# Autodesk Inventor assembly: Hinge
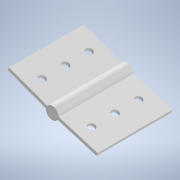
[picture p0: Inventor's stored thumbnail of the model, 180x180]
Saved by Autodesk Inventor 2020 (Build 240168000, 168)
## iProperties
Created: 2021-11-11
Part Number: Hinge
Document SubType Name: Assembly
Designer: 17185
Author: 17185
## Documents named in this file (3)
- C:\Users\17185\Desktop\chassis draft\Hinge\Hinge.iam
- C:\Users\17185\Desktop\chassis draft\Hinge\leaf.ipt
- C:\Users\17185\Desktop\chassis draft\Hinge\Pin.ipt
## Components (3 placed, 2 different names)
1. leaf:1 — Mate:1, Flush:1
2. leaf:2 — Flush:2, Mate:2
3. Pin:1 — Mate:1, Flush:1, Flush:2, Mate:2
## Relationships (4: Mate 2, Flush 2)
- Mate:1: leaf:1 ↔ Pin:1
- Flush:1: leaf:1 ↔ Pin:1
- Flush:2: leaf:2 ↔ Pin:1
- Mate:2: leaf:2 ↔ Pin:1
